# Autodesk Inventor assembly: 下半身
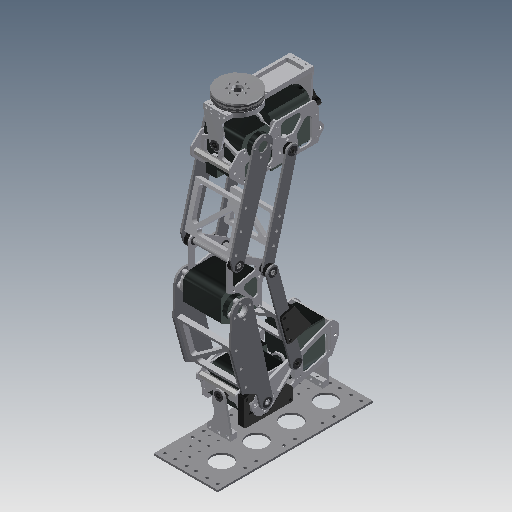
[picture p0: Inventor's stored thumbnail of the model, 512x512]
Saved by Autodesk Inventor 2017.3 (Build 213256000, 256)
## iProperties
Created: 2016-04-27
Part Number: 下半身
Document SubType Name: Assembly
Designer: hiroaki
Mass: 916.815 g
Surface Area: 2246.55 cm^2
Volume: 410.34 cm^3
Density: 2.23428 g/cm^3
Author: hiroaki
## Documents named in this file (12)
- C:\Users\haya\Desktop\GankenKun0_5\下半身.iam
- C:\Users\haya\Desktop\GankenKun0_5\下半身\膝\膝_1_1.iam
- C:\Users\haya\Desktop\GankenKun0_5\下半身\リンク\ふともも\リンク_ふともも_前_1.iam
- C:\Users\haya\Desktop\GankenKun0_5\下半身\リンク\ふともも\リンク_ふともも_後ろ_1.iam
- C:\Users\haya\Desktop\GankenKun0_5\下半身\リンク\ふくらはぎ\リンク_ふくらはぎ_前_1.iam
- C:\Users\haya\Desktop\GankenKun0_5\下半身\リンク\ふくらはぎ\リンク_ふくらはぎ_後ろ_1.iam
- C:\Users\haya\Desktop\GankenKun0_5\下半身\付け根\付け根_1.iam
- C:\Users\haya\Desktop\GankenKun0_5\下半身\足裏\足裏_1_1.iam
- C:\Users\haya\Desktop\GankenKun0_5\下半身\付け根ロール\付け根ロール_1.iam
- C:\Users\haya\Desktop\GankenKun0_5\下半身\足首\足首_1.iam
- C:\Users\haya\Desktop\GankenKun0_5\下半身\足首\足首_独立ピッチ_1.iam
- C:\Users\haya\Desktop\GankenKun0_5\ジグ\ジグ_1_1.ipt
## Components (11 placed, 11 different names)
1. 付け根ロール_1:1 [sub-assembly] — 挿入:23, 挿入:24, 角度:9, 角度:11, 角度:12, 角度:15
2. 膝_1_1:1 [sub-assembly] — 角度:2, 角度:3, 角度:5, 角度:6, 角度:7, 角度:8, 角度:13, 角度:14, 挿入:7, 挿入:8, 挿入:11, 挿入:12, 挿入:35, 挿入:36, 挿入:37, 挿入:38
3. リンク_ふともも_前_1:1 [sub-assembly] — 角度:2, 挿入:3, 挿入:4, 角度:5, 角度:8, 挿入:11, 挿入:12, 角度:13, 角度:17
4. リンク_ふともも_後ろ_1:1 [sub-assembly] — 挿入:5, 挿入:6, 挿入:7, 挿入:8, 挿入:9, 挿入:10, 角度:17
5. リンク_ふくらはぎ_前_1:1 [sub-assembly] — 角度:3, 角度:6, 角度:7, 挿入:33, 挿入:34, 挿入:35, 挿入:36, 挿入:37, 挿入:38, 角度:14, 角度:18
6. リンク_ふくらはぎ_後ろ_1:1 [sub-assembly] — 挿入:5, 挿入:6, 挿入:31, 挿入:32, 角度:18
7. 付け根_1:1 [sub-assembly] — 挿入:3, 挿入:4, 挿入:9, 挿入:10, 挿入:23, 挿入:24, 角度:9, 角度:11, 角度:12, 角度:16, 挿入:39, 挿入:40
8. 足裏_1_1:1 [sub-assembly] — 挿入:27, 挿入:28, 角度:15
9. 足首_1:1 [sub-assembly] — 挿入:27, 挿入:28, 挿入:29, 挿入:30, 角度:16
10. 足首_独立ピッチ_1:1 [sub-assembly] — 挿入:29, 挿入:30, 挿入:31, 挿入:32, 挿入:33, 挿入:34
11. ジグ_1_1:1 — 挿入:39, 挿入:40
## Relationships (41: Insert 26, Angle 15)
- 角度:2 [Angle] (-80 deg): 膝_1_1:1 ↔ リンク_ふともも_前_1:1
- 角度:3 [Angle] (-80 deg): 膝_1_1:1 ↔ リンク_ふくらはぎ_前_1:1
- 挿入:3 [Insert]: リンク_ふともも_前_1:1 ↔ 付け根_1:1
- 挿入:4 [Insert]: リンク_ふともも_前_1:1 ↔ 付け根_1:1
- 角度:5 [Angle] (15 deg): 膝_1_1:1 ↔ リンク_ふともも_前_1:1
- 角度:6 [Angle] (-15 deg): 膝_1_1:1 ↔ リンク_ふくらはぎ_前_1:1
- 角度:7 [Angle] (-30 deg): 膝_1_1:1 ↔ リンク_ふくらはぎ_前_1:1
- 角度:8 [Angle] (-30 deg): 膝_1_1:1 ↔ リンク_ふともも_前_1:1
- 挿入:5 [Insert]: リンク_ふともも_後ろ_1:1 ↔ リンク_ふくらはぎ_後ろ_1:1
- 挿入:6 [Insert]: リンク_ふともも_後ろ_1:1 ↔ リンク_ふくらはぎ_後ろ_1:1
- 角度:13 [Angle] (0 deg): 膝_1_1:1 ↔ リンク_ふともも_前_1:1
- 角度:14 [Angle] (0 deg): 膝_1_1:1 ↔ リンク_ふくらはぎ_前_1:1
- 挿入:7 [Insert]: 膝_1_1:1 ↔ リンク_ふともも_後ろ_1:1
- 挿入:8 [Insert]: 膝_1_1:1 ↔ リンク_ふともも_後ろ_1:1
- 挿入:9 [Insert]: リンク_ふともも_後ろ_1:1 ↔ 付け根_1:1
- 挿入:10 [Insert]: リンク_ふともも_後ろ_1:1 ↔ 付け根_1:1
- 挿入:11 [Insert]: 膝_1_1:1 ↔ リンク_ふともも_前_1:1
- 挿入:12 [Insert]: 膝_1_1:1 ↔ リンク_ふともも_前_1:1
- 挿入:23 [Insert]: 付け根ロール_1:1 ↔ 付け根_1:1
- 挿入:24 [Insert]: 付け根ロール_1:1 ↔ 付け根_1:1
- 角度:9 [Angle] (0 deg): 付け根ロール_1:1 ↔ 付け根_1:1
- 角度:11 [Angle] (20 deg): 付け根ロール_1:1 ↔ 付け根_1:1
- 角度:12 [Angle] (-45 deg): 付け根ロール_1:1 ↔ 付け根_1:1
- 挿入:27 [Insert]: 足裏_1_1:1 ↔ 足首_1:1
- 挿入:28 [Insert]: 足裏_1_1:1 ↔ 足首_1:1
- 挿入:29 [Insert]: 足首_1:1 ↔ 足首_独立ピッチ_1:1
- 挿入:30 [Insert]: 足首_1:1 ↔ 足首_独立ピッチ_1:1
- 挿入:31 [Insert]: リンク_ふくらはぎ_後ろ_1:1 ↔ 足首_独立ピッチ_1:1
- 挿入:32 [Insert]: リンク_ふくらはぎ_後ろ_1:1 ↔ 足首_独立ピッチ_1:1
- 挿入:33 [Insert]: リンク_ふくらはぎ_前_1:1 ↔ 足首_独立ピッチ_1:1
- 挿入:34 [Insert]: リンク_ふくらはぎ_前_1:1 ↔ 足首_独立ピッチ_1:1
- 挿入:35 [Insert]: 膝_1_1:1 ↔ リンク_ふくらはぎ_前_1:1
- 挿入:36 [Insert]: 膝_1_1:1 ↔ リンク_ふくらはぎ_前_1:1
- 挿入:37 [Insert]: 膝_1_1:1 ↔ リンク_ふくらはぎ_前_1:1
- 挿入:38 [Insert]: 膝_1_1:1 ↔ リンク_ふくらはぎ_前_1:1
- 角度:15 [Angle] (0 deg): 付け根ロール_1:1 ↔ 足裏_1_1:1
- 角度:16 [Angle] (0 deg): 付け根_1:1 ↔ 足首_1:1
- 挿入:39 [Insert]: 付け根_1:1 ↔ ジグ_1_1:1
- 挿入:40 [Insert]: 付け根_1:1 ↔ ジグ_1_1:1
- 角度:17 [Angle] (0 deg): リンク_ふともも_前_1:1 ↔ リンク_ふともも_後ろ_1:1
- 角度:18 [Angle] (0 deg): リンク_ふくらはぎ_前_1:1 ↔ リンク_ふくらはぎ_後ろ_1:1
